# Autodesk Inventor assembly: extruder
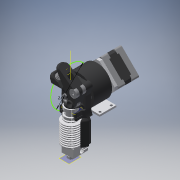
[picture p0: Inventor's stored thumbnail of the model, 180x180]
Saved by Autodesk Inventor 2016 (Build 200138000, 138)
## iProperties
Created: 2016-05-21
Part Number: extruder
Document SubType Name: Assembly
Designer: brent
Author: brent
## Documents named in this file (7)
- C:\Users\brent\OneDrive\personal\printer_cad\extruder\v1\extruder.iam
- C:\Users\brent\OneDrive\personal\printer_cad\extruder\v1\extruder_sketch.ipt
- C:\Users\brent\OneDrive\personal\printer_cad\offtheshelf\gearedstepper.ipt
- C:\Users\brent\OneDrive\personal\printer_cad\offtheshelf\e3dv6.ipt
- C:\Users\brent\OneDrive\personal\printer_cad\offtheshelf\mk8_drivegear.ipt
- C:\Users\brent\OneDrive\personal\printer_cad\offtheshelf\extruder_spring.ipt
- C:\Users\brent\OneDrive\personal\printer_cad\offtheshelf\623bearing.ipt
## Components (8 placed, 6 different names)
1. extruder_sketch:1 — Mate:1, Mate:2, Mate:3, Mate:4, Mate:6, Flush:1, Mate:7, Mate:8, Mate:9, Mate:10, Mate:11, Mate:12, Mate:13, Mate:14
2. gearedstepper:1 — Mate:3, Mate:4, Mate:5, Mate:8
3. e3dv6:1 — Mate:1, Mate:2
4. mk8_drivegear:1 — Mate:5, Mate:6
5. extruder_spring:1 — Flush:1, Mate:7
6. 623bearing:1 — Mate:9, Mate:10
7. 623bearing:2 — Mate:11, Mate:14
8. 623bearing:3 — Mate:12, Mate:13
## Relationships (15: Mate 14, Flush 1)
- Mate:1: extruder_sketch:1 ↔ e3dv6:1
- Mate:2: extruder_sketch:1 ↔ e3dv6:1
- Mate:3: extruder_sketch:1 ↔ gearedstepper:1
- Mate:4: extruder_sketch:1 ↔ gearedstepper:1
- Mate:5: gearedstepper:1 ↔ mk8_drivegear:1
- Mate:6 (-3.35 mm): extruder_sketch:1 ↔ mk8_drivegear:1
- Flush:1: extruder_sketch:1 ↔ extruder_spring:1
- Mate:7: extruder_sketch:1 ↔ extruder_spring:1
- Mate:8: extruder_sketch:1 ↔ gearedstepper:1
- Mate:9: extruder_sketch:1 ↔ 623bearing:1
- Mate:10: extruder_sketch:1 ↔ 623bearing:1
- Mate:11: extruder_sketch:1 ↔ 623bearing:2
- Mate:12: extruder_sketch:1 ↔ 623bearing:3
- Mate:13: extruder_sketch:1 ↔ 623bearing:3
- Mate:14: extruder_sketch:1 ↔ 623bearing:2
